# Autodesk Inventor assembly: MIR_HbSocketU02ForChild
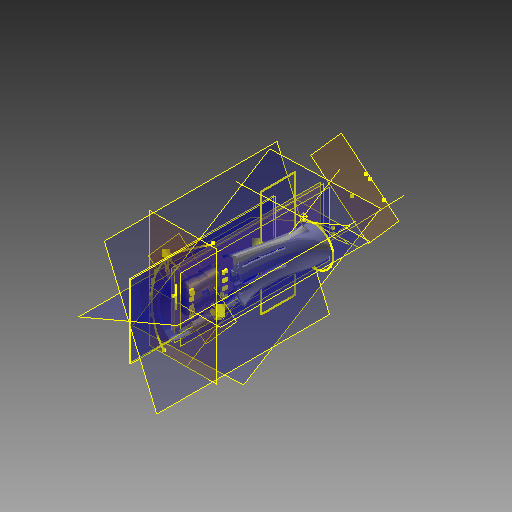
[picture p0: Inventor's stored thumbnail of the model, 512x512]
Saved by Autodesk Inventor 2018 (Build 220112000, 112)
## iProperties
Created: 2015-02-09
Part Number: MIR_HbSocketU02ForChild
Document SubType Name: Assembly
Designer: sktom
Author: Yamaura
## Documents named in this file (10)
- D:\cloudstrage\NextCloud\Cad_mechanical\HACKberry_sktometometo\HACKberry-hardware\3D_69%inlength\Inventor\HbSocketU02ForChild\MIR_HbSocketU02ForChild.iam
- D:\cloudstrage\NextCloud\Cad_mechanical\HACKberry_sktometometo\HACKberry-hardware\3D_69%inlength\Inventor\HbSocketU02ForChild\MIR_HbBatteryDoorKnob03.ipt
- D:\cloudstrage\NextCloud\Cad_mechanical\HACKberry_sktometometo\HACKberry-hardware\3D_69%inlength\Inventor\HbSocketU02ForChild\MIR_HbBatteryHingeC03.ipt
- D:\cloudstrage\NextCloud\Cad_mechanical\HACKberry_sktometometo\HACKberry-hardware\3D_69%inlength\Inventor\HbSocketU02ForChild\MIR_HbBatteryHingeB03.ipt
- D:\cloudstrage\NextCloud\Cad_mechanical\HACKberry_sktometometo\HACKberry-hardware\3D_69%inlength\Inventor\HbSocketU02ForChild\MIR_HbBatteryHingeA03.ipt
- D:\cloudstrage\NextCloud\Cad_mechanical\HACKberry_sktometometo\HACKberry-hardware\3D_69%inlength\Inventor\HbSocketU02ForChild\MIR_HbBatteryDoor03.ipt
- D:\cloudstrage\NextCloud\Cad_mechanical\HACKberry_sktometometo\HACKberry-hardware\3D_69%inlength\Inventor\HbSocketU02ForChild\MIR_HbMainFrameA01.ipt
- D:\cloudstrage\NextCloud\Cad_mechanical\HACKberry_sktometometo\HACKberry-hardware\3D_69%inlength\Inventor\HbSocketU02ForChild\MIR_HbMainFrameB01.ipt
- D:\cloudstrage\NextCloud\Cad_mechanical\HACKberry_sktometometo\HACKberry-hardware\3D_69%inlength\Inventor\HbSocketU02ForChild\MIR_HbBatteryDoorLever03.ipt
- D:\cloudstrage\NextCloud\Cad_mechanical\HACKberry_sktometometo\HACKberry-hardware\3D_69%inlength\Inventor\HbBatteryCase\MIR_HbBatteryCase.iam
## Components (12 placed, 9 different names)
1. MIR_HbBatteryHingeC03:1
2. MIR_HbBatteryHingeB03:1
3. MIR_HbBatteryHingeA03:1
4. MIR_HbBatteryDoor03:1
5. MIR_HbMainFrameA01:1
6. MIR_HbBatteryDoorKnob03:2
7. MIR_HbMainFrameB01:1
8. MIR_HbBatteryCase:1 [sub-assembly]
9. MIR_HbBatteryDoorKnob03:1
10. MIR_HbBatteryDoorKnob03:3
11. MIR_HbBatteryDoorLever03:1
12. MIR_HbBatteryDoorLever03:2
## Component patterns: (2 elements, first: MIR_HbBatteryDoorKnob03:1), (2 elements, first: MIR_HbBatteryDoorLever03:1)
